# Autodesk Inventor assembly: z idler pulley 2
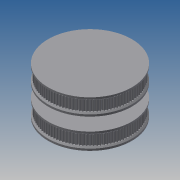
[picture p0: Inventor's stored thumbnail of the model, 180x180]
Saved by Autodesk Inventor 2013 (Build 170138000, 138)
## iProperties
Created: 2017-03-30
Part Number: z idler pulley 2
Document SubType Name: Assembly
Designer: employee
Author: employee
## Documents named in this file (2)
- C:\Users\employee\Desktop\SCARA\z idler pulley 2.iam
- C:\Users\employee\Desktop\SCARA\100 pulley blank.ipt
## Components (2 placed, 1 different names)
1. 100 pulley blank:1 — Insert:1, Mate:1
2. 100 pulley blank:2 — Insert:1, Mate:1
## Relationships (2: Insert 1, Mate 1)
- Insert:1 (10.1 mm): 100 pulley blank:1 ↔ 100 pulley blank:2
- Mate:1: 100 pulley blank:1 ↔ 100 pulley blank:2
